# Autodesk Inventor assembly: 0008-10-04 Z axis
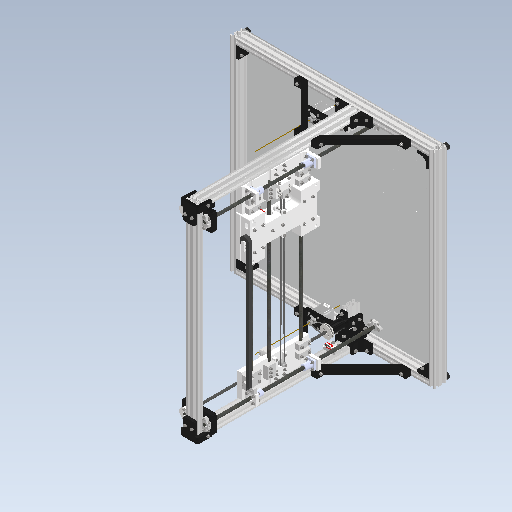
[picture p0: Inventor's stored thumbnail of the model, 512x512]
Saved by Autodesk Inventor 2020 (Build 240168000, 168)
## iProperties
Created: 2021-02-20
Part Number: 0008-10-04 Z axis
Document SubType Name: Assembly
Designer: Iulian Bors
Description: Z axis
Author: Iulian Bors
Subject: 10-04
## Documents named in this file (27)
- Z:\I.A.B\Proiecte\0008 I.A.B 3D 2.1 Imprimanta aracet Metal\10 Mecanic\0008-10-04 Z axis.iam
- Z:\I.A.B\Proiecte\0008 I.A.B 3D 2.1 Imprimanta aracet Metal\10 Mecanic\0008-10-1001 NEMA17 - Motor de passo.ipt
- Z:\I.A.B\Proiecte\0008 I.A.B 3D 2.1 Imprimanta aracet Metal\10 Mecanic\0008-10-1011 GT2 Timing Pulley 20 Tooth.ipt
- Z:\I.A.B\Proiecte\0008 I.A.B 3D 2.1 Imprimanta aracet Metal\10 Mecanic\0008-10-1010 Bara 10.ipt
- Z:\I.A.B\Proiecte\0008 I.A.B 3D 2.1 Imprimanta aracet Metal\10 Mecanic\0008-10-1014 T8 screw.ipt
- Z:\I.A.B\Proiecte\0008 I.A.B 3D 2.1 Imprimanta aracet Metal\10 Mecanic\0008-10-016 Suport Motor Z.ipt
- Z:\I.A.B\Proiecte\0008 I.A.B 3D 2.1 Imprimanta aracet Metal\10 Mecanic\0008-10-1005 ISO 1224-1 - 10 - 8 x 22 x 7.ipt
- Z:\I.A.B\Proiecte\0008 I.A.B 3D 2.1 Imprimanta aracet Metal\10 Mecanic\0008-10-015 roata condusa GT2.ipt
- Z:\I.A.B\Proiecte\0008 I.A.B 3D 2.1 Imprimanta aracet Metal\10 Mecanic\0008-10-1015 Synchronous Belt2.ipt
- Z:\I.A.B\Proiecte\0008 I.A.B 3D 2.1 Imprimanta aracet Metal\10 Mecanic\0008-10-021 Suport Motor Z R.ipt
- Z:\I.A.B\Proiecte\0008 I.A.B 3D 2.1 Imprimanta aracet Metal\10 Mecanic\0008-10-1022 SHF10.ipt
- Z:\I.A.B\Proiecte\0008 I.A.B 3D 2.1 Imprimanta aracet Metal\10 Mecanic\0008-10-034 Suport_Rulment.ipt
- Z:\I.A.B\Proiecte\0008 I.A.B 3D 2.1 Imprimanta aracet Metal\20 Electric\0008-20-1003 Switch.ipt
- Z:\I.A.B\Proiecte\0008 I.A.B 3D 2.1 Imprimanta aracet Metal\10 Mecanic\0008-10-056.ipt
- Z:\I.A.B\Proiecte\0008 I.A.B 3D 2.1 Imprimanta aracet Metal\10 Mecanic\0008-10-01 Sckeleton_Shrinkwrap.ipt
- Z:\I.A.B\Proiecte\0008 I.A.B 3D 2.1 Imprimanta aracet Metal\10 Mecanic\0008-10-2001 DIN 934 - M4 x 0.7.ipt
- Z:\I.A.B\Proiecte\0008 I.A.B 3D 2.1 Imprimanta aracet Metal\10 Mecanic\0008-10-2000 DIN 6912 - M4 x 25.ipt
- Z:\I.A.B\Proiecte\0008 I.A.B 3D 2.1 Imprimanta aracet Metal\10 Mecanic\0008-10-2025 DIN 7984 - M4 x 20.ipt
- Z:\I.A.B\Proiecte\0008 I.A.B 3D 2.1 Imprimanta aracet Metal\10 Mecanic\0008-10-2002 DIN 125 - A 4.3.ipt
- Z:\I.A.B\Proiecte\0008 I.A.B 3D 2.1 Imprimanta aracet Metal\10 Mecanic\SurubM4x35.iam
- Z:\I.A.B\Proiecte\0008 I.A.B 3D 2.1 Imprimanta aracet Metal\10 Mecanic\0008-10-2010 M 5 Canal.ipt
- Z:\I.A.B\Proiecte\0008 I.A.B 3D 2.1 Imprimanta aracet Metal\10 Mecanic\0008-10-2011 DIN 7984 - M5 x 16.ipt
- Z:\I.A.B\Proiecte\0008 I.A.B 3D 2.1 Imprimanta aracet Metal\10 Mecanic\0008-10-2012 DIN 125 - A 5.3.ipt
- Z:\I.A.B\Proiecte\0008 I.A.B 3D 2.1 Imprimanta aracet Metal\10 Mecanic\0008-10-2005 DIN 125 - A 3.2.ipt
- Z:\I.A.B\Proiecte\0008 I.A.B 3D 2.1 Imprimanta aracet Metal\10 Mecanic\0008-10-2006 DIN 7984 - M3 x 16.ipt
- Z:\I.A.B\Proiecte\0008 I.A.B 3D 2.1 Imprimanta aracet Metal\10 Mecanic\0008-10-2026.ipt
- Z:\I.A.B\Proiecte\0008 I.A.B 3D 2.1 Imprimanta aracet Metal\10 Mecanic\0008-10-02 X Axis_Shrinkwrap_1.ipt
## Components (111 placed, 27 different names)
1. 0008-10-1010 Bara 10.ipt:1 — Flush:35, Insert:15, Insert:16
2. 0008-10-1010 Bara 10.ipt:2 — Flush:35, Insert:17, Insert:18, Mate:231
3. 0008-10-1014 T8 screw.ipt:3 — Mate:47, Mate:50, Mate:168
4. 0008-10-1014 T8 screw.ipt:4 — Mate:57, Mate:58, Mate:82, Mate:113, Mate:176, Mate:230
5. 0008-10-021 Suport Motor Z R.ipt:5 — Mate:47, Mate:48, Mate:49, Insert:6, Mate:211, Mate:213, Mate:214, Insert:60, Insert:61, Insert:62, Insert:84, Insert:85, Insert:86, Insert:87
6. 0008-10-1005 ISO 1224-1 - 10 - 8 x 22 x 7.ipt:6 — Insert:4, Insert:6
7. 0008-10-015 roata condusa GT2.ipt:7 — Insert:4, Mate:202, Mate:225, Mate:226
8. 0008-10-1001 NEMA17 - Motor de passo.ipt:8 — Insert:5, Mate:48, Mate:49
9. 0008-10-1011 GT2 Timing Pulley 20 Tooth.ipt:9 — Insert:5, Mate:51, Mate:52
10. 0008-10-1015 Synchronous Belt2.ipt:10 — Mate:50, Mate:51, Mate:52, Mate:202
11. 0008-10-016 Suport Motor Z.ipt:11 — Mate:82, Angle:1, Angle:2, Mate:207, Mate:208, Mate:209, Mate:211, Flush:143, Mate:215, Mate:216, Mate:224, Insert:69, Insert:70, Insert:71, Insert:73, Insert:77, Insert:78, Insert:79
12. 0008-10-1005 ISO 1224-1 - 10 - 8 x 22 x 7.ipt:12
13. 0008-10-015 roata condusa GT2.ipt:13 — Mate:57, Mate:227, Mate:228
14. 0008-10-1001 NEMA17 - Motor de passo.ipt:14 — Mate:113
15. 0008-10-1011 GT2 Timing Pulley 20 Tooth.ipt:15
16. 0008-10-1015 Synchronous Belt2.ipt:16 — Mate:58, Mate:224
17. 0008-10-1022 SHF10.ipt:17 — Insert:16, Flush:140, Mate:220, Mate:221, Insert:25, Insert:33, Insert:37
18. 0008-10-1022 SHF10.ipt:18 — Insert:18, Flush:140, Insert:21, Insert:27, Insert:44, Insert:45, Insert:96
19. 0008-10-1022 SHF10.ipt:19 — Insert:17, Mate:219, Insert:29, Insert:46, Insert:47
20. 0008-10-1022 SHF10.ipt:20 — Insert:15, Mate:222, Insert:24, Insert:50, Insert:51
21. 0008-10-034 Suport_Rulment.ipt:21 — Mate:217, Angle:6, Insert:52, Insert:53
22. 0008-10-1005 ISO 1224-1 - 10 - 8 x 22 x 7.ipt:22 — Mate:168
23. 0008-10-034 Suport_Rulment.ipt:23 — Mate:218, Angle:7, Insert:48, Insert:49
24. 0008-10-1005 ISO 1224-1 - 10 - 8 x 22 x 7.ipt:24 — Mate:176
25. 0008-20-1003 Switch.ipt:25 — Mate:206, Flush:135, Flush:136, Insert:88, Insert:89
26. 0008-10-056.ipt:26 — Mate:206, Flush:135, Flush:136, Mate:223, Flush:144, Insert:94, Insert:95
27. 0008-10-01 Sckeleton_Shrinkwrap.ipt:27 — Flush:143, Mate:213, Mate:214, Mate:215, Mate:216, Mate:217, Angle:6, Mate:218, Angle:7, Insert:21, Mate:219, Mate:220, Mate:221, Mate:222, Mate:223, Flush:144
28. 0008-10-2001 DIN 934 - M4 x 0.7.ipt:28
29. 0008-10-2000 DIN 6912 - M4 x 25.ipt:29 — Insert:24
30. 0008-10-2001 DIN 934 - M4 x 0.7.ipt:30
31. 0008-10-2000 DIN 6912 - M4 x 25.ipt:31 — Insert:25
32. 0008-10-2001 DIN 934 - M4 x 0.7.ipt:32
33. 0008-10-2000 DIN 6912 - M4 x 25.ipt:33 — Insert:27
34. 0008-10-2001 DIN 934 - M4 x 0.7.ipt:34
35. 0008-10-2000 DIN 6912 - M4 x 25.ipt:35 — Insert:29
36. 0008-10-2025 DIN 7984 - M4 x 20.ipt:36 — Insert:30, Insert:31
37. 0008-10-2001 DIN 934 - M4 x 0.7.ipt:37 — Insert:31, Insert:32
38. 0008-10-2002 DIN 125 - A 4.3.ipt:38 — Insert:30, Insert:33
39. 0008-10-2002 DIN 125 - A 4.3.ipt:39 — Insert:32
40. 0008-10-2025 DIN 7984 - M4 x 20.ipt:40
41. 0008-10-2001 DIN 934 - M4 x 0.7.ipt:41
42. 0008-10-2002 DIN 125 - A 4.3.ipt:42 — Insert:37
43. 0008-10-2002 DIN 125 - A 4.3.ipt:43
44. 0008-10-2025 DIN 7984 - M4 x 20.ipt:44
45. 0008-10-2001 DIN 934 - M4 x 0.7.ipt:45
46. 0008-10-2002 DIN 125 - A 4.3.ipt:46 — Insert:44
47. 0008-10-2002 DIN 125 - A 4.3.ipt:47
48. 0008-10-2025 DIN 7984 - M4 x 20.ipt:48 — Mate:229
49. 0008-10-2001 DIN 934 - M4 x 0.7.ipt:49
50. 0008-10-2002 DIN 125 - A 4.3.ipt:50 — Insert:45
51. 0008-10-2002 DIN 125 - A 4.3.ipt:51
52. SurubM4x35.iam:52 [sub-assembly] — Insert:47
53. SurubM4x35.iam:53 [sub-assembly] — Insert:46
54. SurubM4x35.iam:54 [sub-assembly] — Insert:48
55. SurubM4x35.iam:55 [sub-assembly] — Insert:49
56. SurubM4x35.iam:56 [sub-assembly] — Insert:50
57. SurubM4x35.iam:57 [sub-assembly] — Insert:51
58. SurubM4x35.iam:58 [sub-assembly] — Insert:52
59. SurubM4x35.iam:59 [sub-assembly] — Insert:53
60. 0008-10-2010 M 5 Canal.ipt:60
61. 0008-10-2011 DIN 7984 - M5 x 16.ipt:61
62. 0008-10-2012 DIN 125 - A 5.3.ipt:62 — Insert:61
63. 0008-10-2010 M 5 Canal.ipt:63
64. 0008-10-2011 DIN 7984 - M5 x 16.ipt:64
65. 0008-10-2012 DIN 125 - A 5.3.ipt:65 — Insert:60
66. 0008-10-2010 M 5 Canal.ipt:66
67. 0008-10-2011 DIN 7984 - M5 x 16.ipt:67
68. 0008-10-2012 DIN 125 - A 5.3.ipt:68 — Insert:62
69. 0008-10-2010 M 5 Canal.ipt:69
70. 0008-10-2011 DIN 7984 - M5 x 16.ipt:70
71. 0008-10-2012 DIN 125 - A 5.3.ipt:71 — Insert:71
72. 0008-10-2010 M 5 Canal.ipt:72
73. 0008-10-2011 DIN 7984 - M5 x 16.ipt:73
74. 0008-10-2012 DIN 125 - A 5.3.ipt:74 — Insert:70
75. 0008-10-2010 M 5 Canal.ipt:75
76. 0008-10-2011 DIN 7984 - M5 x 16.ipt:76
77. 0008-10-2012 DIN 125 - A 5.3.ipt:77 — Insert:69
78. 0008-10-2005 DIN 125 - A 3.2.ipt:78 — Insert:72, Insert:73
79. 0008-10-2006 DIN 7984 - M3 x 16.ipt:79 — Insert:72
80. 0008-10-2005 DIN 125 - A 3.2.ipt:80 — Insert:79
81. 0008-10-2006 DIN 7984 - M3 x 16.ipt:81
82. 0008-10-2005 DIN 125 - A 3.2.ipt:82 — Insert:78
83. 0008-10-2006 DIN 7984 - M3 x 16.ipt:83
84. 0008-10-2005 DIN 125 - A 3.2.ipt:84 — Insert:77
85. 0008-10-2006 DIN 7984 - M3 x 16.ipt:85
86. 0008-10-2005 DIN 125 - A 3.2.ipt:86 — Insert:84
87. 0008-10-2006 DIN 7984 - M3 x 16.ipt:87
88. 0008-10-2005 DIN 125 - A 3.2.ipt:88 — Insert:85
89. 0008-10-2006 DIN 7984 - M3 x 16.ipt:89
90. 0008-10-2005 DIN 125 - A 3.2.ipt:90 — Insert:86
91. 0008-10-2006 DIN 7984 - M3 x 16.ipt:91
92. 0008-10-2005 DIN 125 - A 3.2.ipt:92 — Insert:87
93. 0008-10-2006 DIN 7984 - M3 x 16.ipt:93
94. 0008-10-2006 DIN 7984 - M3 x 16.ipt:94 — Insert:89
95. 0008-10-2006 DIN 7984 - M3 x 16.ipt:95 — Insert:88
96. 0008-10-2010 M 5 Canal.ipt:96
97. 0008-10-2011 DIN 7984 - M5 x 16.ipt:97
98. 0008-10-2012 DIN 125 - A 5.3.ipt:98 — Insert:95
99. 0008-10-2010 M 5 Canal.ipt:99
100. 0008-10-2011 DIN 7984 - M5 x 16.ipt:100
101. 0008-10-2012 DIN 125 - A 5.3.ipt:101 — Insert:94
102. 0008-10-01 Sckeleton_Shrinkwrap:3 — Insert:96, Mate:229
103. 0008-10-02 X Axis_Shrinkwrap_1:2 — Mate:230, Mate:231
104. 0008-10-2026.ipt:102 — Mate:225, Mate:226
105. 0008-10-2026.ipt:103
106. 0008-10-2026.ipt:104
107. 0008-10-2026.ipt:105
108. 0008-10-2026.ipt:106 — Mate:227, Mate:228
109. 0008-10-2026.ipt:107
110. 0008-10-2026.ipt:108
111. 0008-10-2026.ipt:109
## Component patterns: (4 elements, first: 0008-10-2026.ipt:102), (4 elements, first: 0008-10-2026.ipt:106)
## Relationships (138: Insert 88, Mate 40, Flush 6, Angle 4)
- Flush:35: 0008-10-1010 Bara 10.ipt:1 ↔ 0008-10-1010 Bara 10.ipt:2
- Insert:4: 0008-10-1005 ISO 1224-1 - 10 - 8 x 22 x 7.ipt:6 ↔ 0008-10-015 roata condusa GT2.ipt:7
- Mate:47 (1 mm): 0008-10-1014 T8 screw.ipt:3 ↔ 0008-10-021 Suport Motor Z R.ipt:5
- Insert:5: 0008-10-1001 NEMA17 - Motor de passo.ipt:8 ↔ 0008-10-1011 GT2 Timing Pulley 20 Tooth.ipt:9
- Mate:48: 0008-10-021 Suport Motor Z R.ipt:5 ↔ 0008-10-1001 NEMA17 - Motor de passo.ipt:8
- Mate:49: 0008-10-021 Suport Motor Z R.ipt:5 ↔ 0008-10-1001 NEMA17 - Motor de passo.ipt:8
- Mate:50: 0008-10-1014 T8 screw.ipt:3 ↔ 0008-10-1015 Synchronous Belt2.ipt:10
- Mate:51: 0008-10-1011 GT2 Timing Pulley 20 Tooth.ipt:9 ↔ 0008-10-1015 Synchronous Belt2.ipt:10
- Mate:52 (1.5 mm): 0008-10-1011 GT2 Timing Pulley 20 Tooth.ipt:9 ↔ 0008-10-1015 Synchronous Belt2.ipt:10
- Insert:6: 0008-10-021 Suport Motor Z R.ipt:5 ↔ 0008-10-1005 ISO 1224-1 - 10 - 8 x 22 x 7.ipt:6
- [Insert]: 0008-10-1005 ISO 1224-1 - 10 - 8 x 22 x 7.ipt:12 ↔ 0008-10-015 roata condusa GT2.ipt:13
- [Insert]: 0008-10-1001 NEMA17 - Motor de passo.ipt:14 ↔ 0008-10-1011 GT2 Timing Pulley 20 Tooth.ipt:15
- [Mate]: 0008-10-016 Suport Motor Z.ipt:11 ↔ 0008-10-1001 NEMA17 - Motor de passo.ipt:14
- [Mate]: 0008-10-1011 GT2 Timing Pulley 20 Tooth.ipt:15 ↔ 0008-10-1015 Synchronous Belt2.ipt:16
- [Mate] (1.5 mm): 0008-10-1011 GT2 Timing Pulley 20 Tooth.ipt:15 ↔ 0008-10-1015 Synchronous Belt2.ipt:16
- [Insert]: 0008-10-016 Suport Motor Z.ipt:11 ↔ 0008-10-1005 ISO 1224-1 - 10 - 8 x 22 x 7.ipt:12
- Mate:57: 0008-10-1014 T8 screw.ipt:4 ↔ 0008-10-015 roata condusa GT2.ipt:13
- Mate:58: 0008-10-1014 T8 screw.ipt:4 ↔ 0008-10-1015 Synchronous Belt2.ipt:16
- Mate:82 (1 mm): 0008-10-1014 T8 screw.ipt:4 ↔ 0008-10-016 Suport Motor Z.ipt:11
- Mate:113: 0008-10-1014 T8 screw.ipt:4 ↔ 0008-10-1001 NEMA17 - Motor de passo.ipt:14
- Insert:15: 0008-10-1010 Bara 10.ipt:1 ↔ 0008-10-1022 SHF10.ipt:20
- Insert:16: 0008-10-1010 Bara 10.ipt:1 ↔ 0008-10-1022 SHF10.ipt:17
- Insert:17: 0008-10-1010 Bara 10.ipt:2 ↔ 0008-10-1022 SHF10.ipt:19
- Insert:18: 0008-10-1010 Bara 10.ipt:2 ↔ 0008-10-1022 SHF10.ipt:18
- [Insert]: 0008-10-034 Suport_Rulment.ipt:21 ↔ 0008-10-1005 ISO 1224-1 - 10 - 8 x 22 x 7.ipt:22
- Mate:168: 0008-10-1014 T8 screw.ipt:3 ↔ 0008-10-1005 ISO 1224-1 - 10 - 8 x 22 x 7.ipt:22
- [Insert]: 0008-10-034 Suport_Rulment.ipt:23 ↔ 0008-10-1005 ISO 1224-1 - 10 - 8 x 22 x 7.ipt:24
- Mate:176: 0008-10-1014 T8 screw.ipt:4 ↔ 0008-10-1005 ISO 1224-1 - 10 - 8 x 22 x 7.ipt:24
- Mate:202: 0008-10-015 roata condusa GT2.ipt:7 ↔ 0008-10-1015 Synchronous Belt2.ipt:10
- Mate:206: 0008-20-1003 Switch.ipt:25 ↔ 0008-10-056.ipt:26
- Flush:135: 0008-20-1003 Switch.ipt:25 ↔ 0008-10-056.ipt:26
- Flush:136: 0008-20-1003 Switch.ipt:25 ↔ 0008-10-056.ipt:26
- Angle:1 (180 deg): 0008-10-016 Suport Motor Z.ipt:11
- Angle:2 (0 deg): 0008-10-016 Suport Motor Z.ipt:11
- Mate:207 (267.808 mm): 0008-10-016 Suport Motor Z.ipt:11
- Mate:208 (-68.586 mm): 0008-10-016 Suport Motor Z.ipt:11
- Mate:209 (-40.091 mm): 0008-10-016 Suport Motor Z.ipt:11
- Flush:140: 0008-10-1022 SHF10.ipt:17 ↔ 0008-10-1022 SHF10.ipt:18
- Mate:211 (538.447 mm): 0008-10-021 Suport Motor Z R.ipt:5 ↔ 0008-10-016 Suport Motor Z.ipt:11
- Flush:143 (8.82 mm): 0008-10-016 Suport Motor Z.ipt:11 ↔ 0008-10-01 Sckeleton_Shrinkwrap.ipt:27
- Mate:213: 0008-10-021 Suport Motor Z R.ipt:5 ↔ 0008-10-01 Sckeleton_Shrinkwrap.ipt:27
- Mate:214: 0008-10-021 Suport Motor Z R.ipt:5 ↔ 0008-10-01 Sckeleton_Shrinkwrap.ipt:27
- Mate:215: 0008-10-016 Suport Motor Z.ipt:11 ↔ 0008-10-01 Sckeleton_Shrinkwrap.ipt:27
- Mate:216: 0008-10-016 Suport Motor Z.ipt:11 ↔ 0008-10-01 Sckeleton_Shrinkwrap.ipt:27
- Mate:217: 0008-10-034 Suport_Rulment.ipt:21 ↔ 0008-10-01 Sckeleton_Shrinkwrap.ipt:27
- Angle:6 (180 deg): 0008-10-034 Suport_Rulment.ipt:21 ↔ 0008-10-01 Sckeleton_Shrinkwrap.ipt:27
- Mate:218: 0008-10-034 Suport_Rulment.ipt:23 ↔ 0008-10-01 Sckeleton_Shrinkwrap.ipt:27
- Angle:7 (180 deg): 0008-10-034 Suport_Rulment.ipt:23 ↔ 0008-10-01 Sckeleton_Shrinkwrap.ipt:27
- Insert:21: 0008-10-1022 SHF10.ipt:18 ↔ 0008-10-01 Sckeleton_Shrinkwrap.ipt:27
- Mate:219: 0008-10-1022 SHF10.ipt:19 ↔ 0008-10-01 Sckeleton_Shrinkwrap.ipt:27
- Mate:220: 0008-10-1022 SHF10.ipt:17 ↔ 0008-10-01 Sckeleton_Shrinkwrap.ipt:27
- Mate:221: 0008-10-1022 SHF10.ipt:17 ↔ 0008-10-01 Sckeleton_Shrinkwrap.ipt:27
- Mate:222: 0008-10-1022 SHF10.ipt:20 ↔ 0008-10-01 Sckeleton_Shrinkwrap.ipt:27
- Mate:223: 0008-10-056.ipt:26 ↔ 0008-10-01 Sckeleton_Shrinkwrap.ipt:27
- Flush:144: 0008-10-056.ipt:26 ↔ 0008-10-01 Sckeleton_Shrinkwrap.ipt:27
- Mate:224: 0008-10-016 Suport Motor Z.ipt:11 ↔ 0008-10-1015 Synchronous Belt2.ipt:16
- [Insert]: 0008-10-2001 DIN 934 - M4 x 0.7.ipt:28 ↔ 0008-10-2000 DIN 6912 - M4 x 25.ipt:29
- [Insert]: 0008-10-2001 DIN 934 - M4 x 0.7.ipt:30 ↔ 0008-10-2000 DIN 6912 - M4 x 25.ipt:31
- Insert:24: 0008-10-1022 SHF10.ipt:20 ↔ 0008-10-2000 DIN 6912 - M4 x 25.ipt:29
- Insert:25: 0008-10-1022 SHF10.ipt:17 ↔ 0008-10-2000 DIN 6912 - M4 x 25.ipt:31
- [Insert]: 0008-10-2001 DIN 934 - M4 x 0.7.ipt:32 ↔ 0008-10-2000 DIN 6912 - M4 x 25.ipt:33
- Insert:27: 0008-10-1022 SHF10.ipt:18 ↔ 0008-10-2000 DIN 6912 - M4 x 25.ipt:33
- [Insert]: 0008-10-2001 DIN 934 - M4 x 0.7.ipt:34 ↔ 0008-10-2000 DIN 6912 - M4 x 25.ipt:35
- Insert:29: 0008-10-1022 SHF10.ipt:19 ↔ 0008-10-2000 DIN 6912 - M4 x 25.ipt:35
- Insert:30: 0008-10-2025 DIN 7984 - M4 x 20.ipt:36 ↔ 0008-10-2002 DIN 125 - A 4.3.ipt:38
- Insert:31: 0008-10-2025 DIN 7984 - M4 x 20.ipt:36 ↔ 0008-10-2001 DIN 934 - M4 x 0.7.ipt:37
- Insert:32: 0008-10-2001 DIN 934 - M4 x 0.7.ipt:37 ↔ 0008-10-2002 DIN 125 - A 4.3.ipt:39
- Insert:33: 0008-10-1022 SHF10.ipt:17 ↔ 0008-10-2002 DIN 125 - A 4.3.ipt:38
- [Insert]: 0008-10-2025 DIN 7984 - M4 x 20.ipt:40 ↔ 0008-10-2002 DIN 125 - A 4.3.ipt:42
- [Insert]: 0008-10-2025 DIN 7984 - M4 x 20.ipt:40 ↔ 0008-10-2001 DIN 934 - M4 x 0.7.ipt:41
- [Insert]: 0008-10-2001 DIN 934 - M4 x 0.7.ipt:41 ↔ 0008-10-2002 DIN 125 - A 4.3.ipt:43
- Insert:37: 0008-10-1022 SHF10.ipt:17 ↔ 0008-10-2002 DIN 125 - A 4.3.ipt:42
- [Insert]: 0008-10-2025 DIN 7984 - M4 x 20.ipt:44 ↔ 0008-10-2002 DIN 125 - A 4.3.ipt:46
- [Insert]: 0008-10-2025 DIN 7984 - M4 x 20.ipt:44 ↔ 0008-10-2001 DIN 934 - M4 x 0.7.ipt:45
- [Insert]: 0008-10-2001 DIN 934 - M4 x 0.7.ipt:45 ↔ 0008-10-2002 DIN 125 - A 4.3.ipt:47
- [Insert]: 0008-10-2025 DIN 7984 - M4 x 20.ipt:48 ↔ 0008-10-2002 DIN 125 - A 4.3.ipt:50
- [Insert]: 0008-10-2025 DIN 7984 - M4 x 20.ipt:48 ↔ 0008-10-2001 DIN 934 - M4 x 0.7.ipt:49
- [Insert]: 0008-10-2001 DIN 934 - M4 x 0.7.ipt:49 ↔ 0008-10-2002 DIN 125 - A 4.3.ipt:51
- Insert:44: 0008-10-1022 SHF10.ipt:18 ↔ 0008-10-2002 DIN 125 - A 4.3.ipt:46
- Insert:45: 0008-10-1022 SHF10.ipt:18 ↔ 0008-10-2002 DIN 125 - A 4.3.ipt:50
- Insert:46: 0008-10-1022 SHF10.ipt:19 ↔ SurubM4x35.iam:53
- Insert:47: 0008-10-1022 SHF10.ipt:19 ↔ SurubM4x35.iam:52
- Insert:48: 0008-10-034 Suport_Rulment.ipt:23 ↔ SurubM4x35.iam:54
- Insert:49: 0008-10-034 Suport_Rulment.ipt:23 ↔ SurubM4x35.iam:55
- Insert:50: 0008-10-1022 SHF10.ipt:20 ↔ SurubM4x35.iam:56
- Insert:51: 0008-10-1022 SHF10.ipt:20 ↔ SurubM4x35.iam:57
- Insert:52: 0008-10-034 Suport_Rulment.ipt:21 ↔ SurubM4x35.iam:58
- Insert:53: 0008-10-034 Suport_Rulment.ipt:21 ↔ SurubM4x35.iam:59
- [Insert] (-5 mm): 0008-10-2010 M 5 Canal.ipt:60 ↔ 0008-10-2011 DIN 7984 - M5 x 16.ipt:61
- [Insert]: 0008-10-2011 DIN 7984 - M5 x 16.ipt:61 ↔ 0008-10-2012 DIN 125 - A 5.3.ipt:62
- [Insert] (-5 mm): 0008-10-2010 M 5 Canal.ipt:63 ↔ 0008-10-2011 DIN 7984 - M5 x 16.ipt:64
- [Insert]: 0008-10-2011 DIN 7984 - M5 x 16.ipt:64 ↔ 0008-10-2012 DIN 125 - A 5.3.ipt:65
- [Insert] (-5 mm): 0008-10-2010 M 5 Canal.ipt:66 ↔ 0008-10-2011 DIN 7984 - M5 x 16.ipt:67
- [Insert]: 0008-10-2011 DIN 7984 - M5 x 16.ipt:67 ↔ 0008-10-2012 DIN 125 - A 5.3.ipt:68
- Insert:60: 0008-10-021 Suport Motor Z R.ipt:5 ↔ 0008-10-2012 DIN 125 - A 5.3.ipt:65
- Insert:61: 0008-10-021 Suport Motor Z R.ipt:5 ↔ 0008-10-2012 DIN 125 - A 5.3.ipt:62
- Insert:62: 0008-10-021 Suport Motor Z R.ipt:5 ↔ 0008-10-2012 DIN 125 - A 5.3.ipt:68
- [Insert] (-5 mm): 0008-10-2010 M 5 Canal.ipt:69 ↔ 0008-10-2011 DIN 7984 - M5 x 16.ipt:70
- [Insert]: 0008-10-2011 DIN 7984 - M5 x 16.ipt:70 ↔ 0008-10-2012 DIN 125 - A 5.3.ipt:71
- [Insert] (-5 mm): 0008-10-2010 M 5 Canal.ipt:72 ↔ 0008-10-2011 DIN 7984 - M5 x 16.ipt:73
- [Insert]: 0008-10-2011 DIN 7984 - M5 x 16.ipt:73 ↔ 0008-10-2012 DIN 125 - A 5.3.ipt:74
- [Insert] (-5 mm): 0008-10-2010 M 5 Canal.ipt:75 ↔ 0008-10-2011 DIN 7984 - M5 x 16.ipt:76
- [Insert]: 0008-10-2011 DIN 7984 - M5 x 16.ipt:76 ↔ 0008-10-2012 DIN 125 - A 5.3.ipt:77
- Insert:69: 0008-10-016 Suport Motor Z.ipt:11 ↔ 0008-10-2012 DIN 125 - A 5.3.ipt:77
- Insert:70: 0008-10-016 Suport Motor Z.ipt:11 ↔ 0008-10-2012 DIN 125 - A 5.3.ipt:74
- Insert:71: 0008-10-016 Suport Motor Z.ipt:11 ↔ 0008-10-2012 DIN 125 - A 5.3.ipt:71
- Insert:72: 0008-10-2005 DIN 125 - A 3.2.ipt:78 ↔ 0008-10-2006 DIN 7984 - M3 x 16.ipt:79
- Insert:73: 0008-10-016 Suport Motor Z.ipt:11 ↔ 0008-10-2005 DIN 125 - A 3.2.ipt:78
- [Insert]: 0008-10-2005 DIN 125 - A 3.2.ipt:80 ↔ 0008-10-2006 DIN 7984 - M3 x 16.ipt:81
- [Insert]: 0008-10-2005 DIN 125 - A 3.2.ipt:82 ↔ 0008-10-2006 DIN 7984 - M3 x 16.ipt:83
- [Insert]: 0008-10-2005 DIN 125 - A 3.2.ipt:84 ↔ 0008-10-2006 DIN 7984 - M3 x 16.ipt:85
- Insert:77: 0008-10-016 Suport Motor Z.ipt:11 ↔ 0008-10-2005 DIN 125 - A 3.2.ipt:84
- Insert:78: 0008-10-016 Suport Motor Z.ipt:11 ↔ 0008-10-2005 DIN 125 - A 3.2.ipt:82
- Insert:79: 0008-10-016 Suport Motor Z.ipt:11 ↔ 0008-10-2005 DIN 125 - A 3.2.ipt:80
- [Insert]: 0008-10-2005 DIN 125 - A 3.2.ipt:86 ↔ 0008-10-2006 DIN 7984 - M3 x 16.ipt:87
- [Insert]: 0008-10-2005 DIN 125 - A 3.2.ipt:88 ↔ 0008-10-2006 DIN 7984 - M3 x 16.ipt:89
- [Insert]: 0008-10-2005 DIN 125 - A 3.2.ipt:90 ↔ 0008-10-2006 DIN 7984 - M3 x 16.ipt:91
- [Insert]: 0008-10-2005 DIN 125 - A 3.2.ipt:92 ↔ 0008-10-2006 DIN 7984 - M3 x 16.ipt:93
- Insert:84: 0008-10-021 Suport Motor Z R.ipt:5 ↔ 0008-10-2005 DIN 125 - A 3.2.ipt:86
- Insert:85: 0008-10-021 Suport Motor Z R.ipt:5 ↔ 0008-10-2005 DIN 125 - A 3.2.ipt:88
- Insert:86: 0008-10-021 Suport Motor Z R.ipt:5 ↔ 0008-10-2005 DIN 125 - A 3.2.ipt:90
- Insert:87: 0008-10-021 Suport Motor Z R.ipt:5 ↔ 0008-10-2005 DIN 125 - A 3.2.ipt:92
- Insert:88: 0008-20-1003 Switch.ipt:25 ↔ 0008-10-2006 DIN 7984 - M3 x 16.ipt:95
- Insert:89: 0008-20-1003 Switch.ipt:25 ↔ 0008-10-2006 DIN 7984 - M3 x 16.ipt:94
- [Insert] (-5 mm): 0008-10-2010 M 5 Canal.ipt:96 ↔ 0008-10-2011 DIN 7984 - M5 x 16.ipt:97
- [Insert]: 0008-10-2011 DIN 7984 - M5 x 16.ipt:97 ↔ 0008-10-2012 DIN 125 - A 5.3.ipt:98
- [Insert] (-5 mm): 0008-10-2010 M 5 Canal.ipt:99 ↔ 0008-10-2011 DIN 7984 - M5 x 16.ipt:100
- [Insert]: 0008-10-2011 DIN 7984 - M5 x 16.ipt:100 ↔ 0008-10-2012 DIN 125 - A 5.3.ipt:101
- Insert:94: 0008-10-056.ipt:26 ↔ 0008-10-2012 DIN 125 - A 5.3.ipt:101
- Insert:95: 0008-10-056.ipt:26 ↔ 0008-10-2012 DIN 125 - A 5.3.ipt:98
- Mate:225: 0008-10-015 roata condusa GT2.ipt:7 ↔ 0008-10-2026.ipt:102
- Mate:226: 0008-10-015 roata condusa GT2.ipt:7 ↔ 0008-10-2026.ipt:102
- Mate:227: 0008-10-015 roata condusa GT2.ipt:13 ↔ 0008-10-2026.ipt:106
- Mate:228: 0008-10-015 roata condusa GT2.ipt:13 ↔ 0008-10-2026.ipt:106
- Insert:96: 0008-10-1022 SHF10.ipt:18 ↔ 0008-10-01 Sckeleton_Shrinkwrap:3
- Mate:229: 0008-10-2025 DIN 7984 - M4 x 20.ipt:48 ↔ 0008-10-01 Sckeleton_Shrinkwrap:3
- Mate:230: 0008-10-1014 T8 screw.ipt:4 ↔ 0008-10-02 X Axis_Shrinkwrap_1:2
- Mate:231: 0008-10-1010 Bara 10.ipt:2 ↔ 0008-10-02 X Axis_Shrinkwrap_1:2
## Named parameters: d120_d113 = 0 mm, d121_d114 = 0 mm, d123_d117 = 0 mm, d124_d118 = 1.5 mm, d125_d119 = 0 mm, d126_d110 = 0 mm, d349_d82 = 0 mm, d358_d349_d82 = 0 mm, d92_d88 = 0 mm, d508_d92_d88 = 0 mm, d511_d92_d88 = 0 mm, d513_d92_d88 = 0 mm, d519_d516 = 0 mm, d520_d517 = 0 mm, d521_d515 = 0 mm, d523_d516 = 0 mm, d524_d517 = 0 mm, d525_d515 = 0 mm, d526_d516 = 0 mm, d527_d517 = 0 mm, d528_d515 = 0 mm, d555_d455 = -5 mm, d556_d456 = 0 mm, d541_d555_d455 = -5 mm, d542_d556_d456 = 0 mm, d543_d555_d455 = -5 mm, d544_d556_d456 = 0 mm, d548_d555_d455 = -5 mm, d549_d556_d456 = 0 mm, d550_d555_d455 = -5 mm, d551_d556_d456 = 0 mm, d552_d555_d455 = -5 mm, d553_d556_d456 = 0 mm, d559_d557 = 0 mm, d560_d557 = 0 mm, d561_d557 = 0 mm, d565_d557 = 0 mm, d566_d557 = 0 mm, d567_d557 = 0 mm, d568_d557 = 0 mm, d575_d555_d455 = -5 mm, d576_d556_d456 = 0 mm, d577_d555_d455 = -5 mm, d578_d556_d456 = 0 mm
